# Autodesk Inventor assembly: modularRICH
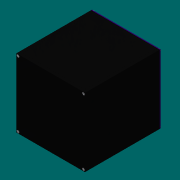
[picture p0: Inventor's stored thumbnail of the model, 180x180]
Saved by Autodesk Inventor 2016 (Build 200138000, 138)
## iProperties
Created: 2015-10-13
Part Number: modularRICH
Document SubType Name: Assembly
Designer: Sawaiz
Author: Sawaiz
## Documents named in this file (10)
- C:\Users\sawaiz\oneDrive\projects\modularRICH\modularRICH.iam
- C:\Users\sawaiz\oneDrive\projects\modularRICH\frame\frame.iam
- C:\Users\sawaiz\oneDrive\projects\modularRICH\fresnelLens.ipt
- C:\Users\sawaiz\oneDrive\projects\modularRICH\mirror\mirrorHolder.iam
- C:\Users\sawaiz\oneDrive\projects\modularRICH\aerogel.ipt
- C:\Users\sawaiz\oneDrive\projects\modularRICH\aerogelHolder.ipt
- C:\Users\sawaiz\oneDrive\projects\modularRICH\detector\fourPmtDetector.iam
- C:\Users\sawaiz\oneDrive\projects\modularRICH\hardware\4-40x0.5in-flat.ipt
- C:\Users\sawaiz\oneDrive\projects\modularRICH\hardware\4-40x0.5in-pan.ipt
- C:\Users\sawaiz\oneDrive\projects\modularRICH\modularRICH.xlsx
## Components (14 placed, 8 different names)
1. frame:1 [sub-assembly] — Angle:1, Mate:3, Mate:4, Mate:5, Mate:6, Mate:7, Mate:8, Flush:2, Mate:10, Mate:11, Flush:3, Flush:4, Mate:12, Mate:13, Flush:5, Mate:14, Mate:15, Mate:16, Flush:6, Flush:7, Flush:8
2. mirrorHolder:1 [sub-assembly] — Flush:2, Mate:10, Mate:11
3. fresnelLens:1 — Mate:4, Mate:5, Mate:6, Mate:9
4. aerogel:1 — Mate:1, Mate:2, Flush:1
5. aerogelHolder:1 — Angle:1, Mate:1, Mate:2, Flush:1, Mate:3, Mate:7, Mate:8, Mate:9
6. fourPmtDetector:1 [sub-assembly] — Flush:3, Flush:4, Mate:12, Mate:17, Mate:18, Mate:19, Mate:20, Mate:21
7. 4-40x0.5in-flat:1 — Mate:13, Flush:5
8. 4-40x0.5in-flat:2 — Mate:14, Flush:8
9. 4-40x0.5in-flat:3 — Mate:16, Flush:6
10. 4-40x0.5in-flat:4 — Mate:15, Flush:7
11. 4-40x0.5in-pan:1 — Mate:17, Flush:11
12. 4-40x0.5in-pan:2 — Flush:10, Flush:11, Mate:18, Mate:19
13. 4-40x0.5in-pan:3 — Flush:9, Flush:10, Mate:20
14. 4-40x0.5in-pan:4 — Flush:9, Mate:21
## Relationships (33: Mate 21, Flush 11, Angle 1)
- Angle:1 (0 deg): frame:1 ↔ aerogelHolder:1
- Mate:1: aerogel:1 ↔ aerogelHolder:1
- Mate:2: aerogel:1 ↔ aerogelHolder:1
- Flush:1: aerogel:1 ↔ aerogelHolder:1
- Mate:3: frame:1 ↔ aerogelHolder:1
- Mate:4: frame:1 ↔ fresnelLens:1
- Mate:5: frame:1 ↔ fresnelLens:1
- Mate:6: frame:1 ↔ fresnelLens:1
- Mate:7: frame:1 ↔ aerogelHolder:1
- Mate:8: frame:1 ↔ aerogelHolder:1
- Mate:9: fresnelLens:1 ↔ aerogelHolder:1
- Flush:2: frame:1 ↔ mirrorHolder:1
- Mate:10: frame:1 ↔ mirrorHolder:1
- Mate:11: frame:1 ↔ mirrorHolder:1
- Flush:3: frame:1 ↔ fourPmtDetector:1
- Flush:4: frame:1 ↔ fourPmtDetector:1
- Mate:12: frame:1 ↔ fourPmtDetector:1
- Mate:13: frame:1 ↔ 4-40x0.5in-flat:1
- Flush:5: frame:1 ↔ 4-40x0.5in-flat:1
- Mate:14: frame:1 ↔ 4-40x0.5in-flat:2
- Mate:15: frame:1 ↔ 4-40x0.5in-flat:4
- Mate:16: frame:1 ↔ 4-40x0.5in-flat:3
- Flush:6: frame:1 ↔ 4-40x0.5in-flat:3
- Flush:7: frame:1 ↔ 4-40x0.5in-flat:4
- Flush:8: frame:1 ↔ 4-40x0.5in-flat:2
- Mate:17: fourPmtDetector:1 ↔ 4-40x0.5in-pan:1
- Flush:9: 4-40x0.5in-pan:3 ↔ 4-40x0.5in-pan:4
- Flush:10: 4-40x0.5in-pan:2 ↔ 4-40x0.5in-pan:3
- Flush:11: 4-40x0.5in-pan:1 ↔ 4-40x0.5in-pan:2
- Mate:18: fourPmtDetector:1 ↔ 4-40x0.5in-pan:2
- Mate:19: fourPmtDetector:1 ↔ 4-40x0.5in-pan:2
- Mate:20: fourPmtDetector:1 ↔ 4-40x0.5in-pan:3
- Mate:21: fourPmtDetector:1 ↔ 4-40x0.5in-pan:4
## Named parameters: acrylicThickness = 6.35 mm, aerogelThickness = 30 mm, height = 127 mm, width = 127 mm, depth = 146.05 mm, mirrorAngle = 5 deg, detectorWidth = 52 mm, detectorHeight = 52 mm, mirrorThickness = 3.175 mm, fresnelThickness = 0.1 mm, grooveDensity = 100, focalLength = 76.2 mm, ior = 1.49, centerThickness = 1.524 mm, fresnelAngle = 90 deg, fresnelEffectiveDiameter = 152.4 mm, mirrorSuppourtWidth = 38.1 mm, backGrooveBit = 4.8006 mm, sensorHolderWidth = 88.9 mm, sensorHolderSesnorHeight = 53.975 mm, sensorHolderSensorWidth = 53.975 mm, sensorHolderHeight = 88.9 mm, sensorHolderSensorHeight = 53.975 mm, sensorHolderORingGroove = 3.175 mm, sensorHolderORing = 3.175 mm, sensorHolderFlushORingID = 304.8 mm, sensorHolderFlushORing = 3.175 mm, oRingWidth = 1.5875 mm, sensorHolderORingID = 203.2 mm, frontBackORingID = 419.1 mm, topBottomHorizontalMirrorGroove = 12.7 mm, backMirrorGroove = 6.35 mm, mirrorGroove = 19.05 mm, compressionPercent = 40, fresnelChamfer = 6.35 mm, mirrorGrooveFillet = 6.35 mm, mirrorGrooveDrill = 6.35 mm, mirrorGrooveMill = 3.175 mm, fresnelMirrorChamfer = 6.35 mm, detectorOpeningHeight = 76.2 mm, detectorOpeningWidth = 76.2 mm, sensorHolderDepth = 19.05 mm, aerogelHeight = 110 mm, aerogelWidth = 110 mm, frameAcrylicThickness = 9.525 mm, internalAcrylicThicnkess = 6.35 mm, internalAcrylicThickness = 6.35 mm, aerogelClearence = 3.175 mm, backplanePCBWidth = 76.2 mm, backplanePCBHeight = 76.2 mm, backplaneHoleOffsett = 6.35 mm, backplanePostionOffsett = 12.7 mm, moduleSlotClearence = 0.79375 mm, testMountWidth = 300 mm, testMountHeight = 300 mm, testMountLength = 500 mm, aerogelHolderDepth = 37.30625 mm, plasticThickness = 6.35 mm
